# Autodesk Inventor assembly: Assembly1
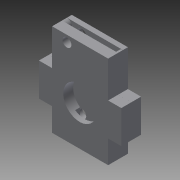
[picture p0: Inventor's stored thumbnail of the model, 180x180]
Saved by Autodesk Inventor 2015 SP1 (Build 190203100, 203)
## iProperties
Created: 2015-06-09
Part Number: Assembly1
Document SubType Name: Assembly
Designer: pc
Author: pc
## Documents named in this file (4)
- C:\Users\pc\Desktop\sensores.diametro\Assembly1.iam
- C:\Users\pc\Desktop\sensores.diametro\soporte.ipt
- C:\Users\pc\Desktop\sensores.diametro\tapa.ipt
- C:\Users\pc\Desktop\sensores.diametro\sensores.ipt
## Components (3 placed, 3 different names)
1. soporte:1 — Flush:1, Flush:2, Mate:2, Mate:3, Mate:4
2. tapa:1 — Flush:1, Flush:2
3. sensores:1 — Mate:2, Mate:3, Mate:4
## Relationships (5: Mate 3, Flush 2)
- Flush:1: soporte:1 ↔ tapa:1
- Flush:2: soporte:1 ↔ tapa:1
- Mate:2: soporte:1 ↔ sensores:1
- Mate:3 (0.5 mm): soporte:1 ↔ sensores:1
- Mate:4: soporte:1 ↔ sensores:1
